# Autodesk Inventor assembly: AddOn_Module
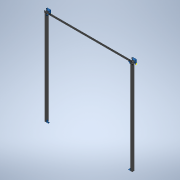
[picture p0: Inventor's stored thumbnail of the model, 180x180]
Saved by Autodesk Inventor 2021 (Build 250183000, 183)
## iProperties
Created: 2021-04-05
Part Number: AddOn_Module
Document SubType Name: Assembly
Designer: Jorian Brusind
Author: Jorian Brusind
## Documents named in this file (5)
- C:\Users\Jorian Brusind\Documents\GitHub\PersonalProjects\HyperRail\Inventor Files\AddOn_Module.iam
- C:\Users\Jorian Brusind\Documents\GitHub\PersonalProjects\Inventor Projects\Useful models\8020_Sets\IPT_20_Series\IPT_20_Series\20-4040_2m.ipt
- C:\Users\Jorian Brusind\Documents\GitHub\PersonalProjects\Inventor Projects\Useful models\8020_Sets\IPT_20_Series\IPT_20_Series\20-2020_variable.ipt
- C:\Users\Jorian Brusind\Documents\GitHub\PersonalProjects\HyperRail\Inventor Files\RightAngle_Bracket.ipt
- C:\Users\Jorian Brusind\Documents\GitHub\PersonalProjects\HyperRail\Inventor Files\Bottom_Stand.ipt
## Components (9 placed, 4 different names)
1. 20-4040_2m:1 — Mate:1, Flush:1, Flush:4, Mate:3, Mate:4, Mate:5, Mate:6, Flush:5, Flush:9, Mate:14, Flush:10
2. 20-4040_2m:2 — Mate:2, Flush:2, Flush:3, Mate:8, Mate:9, Mate:10, Mate:11, Mate:13, Flush:7, Flush:8
3. 20-2020_variable:1 — Mate:1, Flush:1, Mate:2, Flush:2, Flush:3, Flush:4, Mate:7, Mate:12, Flush:6
4. RightAngle_Bracket:1 — Mate:6, Mate:7, Flush:5
5. RightAngle_Bracket:2 — Mate:11, Mate:12, Flush:6
6. RightAngle_Bracket:3 — Flush:9, Mate:14, Flush:10
7. RightAngle_Bracket:4 — Mate:13, Flush:7, Flush:8
8. Bottom_Stand:1 — Mate:3, Mate:4, Mate:5
9. Bottom_Stand:2 — Mate:8, Mate:9, Mate:10
## Relationships (24: Mate 14, Flush 10)
- Mate:1: 20-4040_2m:1 ↔ 20-2020_variable:1
- Flush:1: 20-4040_2m:1 ↔ 20-2020_variable:1
- Mate:2: 20-4040_2m:2 ↔ 20-2020_variable:1
- Flush:2: 20-4040_2m:2 ↔ 20-2020_variable:1
- Flush:3: 20-4040_2m:2 ↔ 20-2020_variable:1
- Flush:4: 20-4040_2m:1 ↔ 20-2020_variable:1
- Mate:3: 20-4040_2m:1 ↔ Bottom_Stand:1
- Mate:4: 20-4040_2m:1 ↔ Bottom_Stand:1
- Mate:5: 20-4040_2m:1 ↔ Bottom_Stand:1
- Mate:6: 20-4040_2m:1 ↔ RightAngle_Bracket:1
- Mate:7: 20-2020_variable:1 ↔ RightAngle_Bracket:1
- Flush:5: 20-4040_2m:1 ↔ RightAngle_Bracket:1
- Mate:8: 20-4040_2m:2 ↔ Bottom_Stand:2
- Mate:9: 20-4040_2m:2 ↔ Bottom_Stand:2
- Mate:10: 20-4040_2m:2 ↔ Bottom_Stand:2
- Mate:11: 20-4040_2m:2 ↔ RightAngle_Bracket:2
- Mate:12: 20-2020_variable:1 ↔ RightAngle_Bracket:2
- Flush:6: 20-2020_variable:1 ↔ RightAngle_Bracket:2
- Mate:13: 20-4040_2m:2 ↔ RightAngle_Bracket:4
- Flush:7: 20-4040_2m:2 ↔ RightAngle_Bracket:4
- Flush:8: 20-4040_2m:2 ↔ RightAngle_Bracket:4
- Flush:9: 20-4040_2m:1 ↔ RightAngle_Bracket:3
- Mate:14: 20-4040_2m:1 ↔ RightAngle_Bracket:3
- Flush:10: 20-4040_2m:1 ↔ RightAngle_Bracket:3
